# Autodesk Inventor assembly: Catapult Launcher
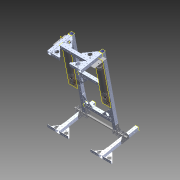
[picture p0: Inventor's stored thumbnail of the model, 180x180]
Saved by Autodesk Inventor 2014 (Build 180170000, 170)
## iProperties
Created: 2014-01-17
Part Number: Catapult Launcher
Document SubType Name: Assembly
Designer: Andrew Toennies
Mass: 1552.27 g
Surface Area: 5150.08 cm^2
Volume: 383.1 cm^3
Density: 4.05187 g/cm^3
Author: Andrew Toennies
## Documents named in this file (14)
- C:\Users\Andrew Toennies\Documents\GitHub\2014buildCAD\New Shooter\Catapult Launcher.iam
- C:\Users\Andrew Toennies\Documents\GitHub\2014buildCAD\New Shooter\Vex Pro 1x1 rectangular tubing 7 in length.ipt
- C:\Users\Andrew Toennies\Documents\GitHub\2014buildCAD\New Shooter\Vex Pro Side Bearing Gusset - OUT OF STOCK 1192014.ipt
- C:\Users\Andrew Toennies\Documents\GitHub\2014buildCAD\New Shooter\Vex Pro Corner Gusset - IN STOCK 1192014.ipt
- C:\Users\Andrew Toennies\Documents\GitHub\2014buildCAD\New Shooter\Bearing ID 0.500 Hex OD 1.125.ipt
- C:\Users\Andrew Toennies\Documents\GitHub\2014buildCAD\New Shooter\Shaft (Steel 0.500 Hex).ipt
- C:\Users\Andrew Toennies\Documents\GitHub\2014buildCAD\New Shooter\Vex Pro 1x1 rectangular tubing 27 in length.ipt
- C:\Users\Andrew Toennies\Documents\GitHub\2014buildCAD\New Shooter\Vex Pro 1x1 rectangular tubing 3 in length.ipt
- C:\Users\Andrew Toennies\Documents\GitHub\2014buildCAD\New Shooter\Vex Pro 1x1 rectangular tubing 11 in length.ipt
- C:\Users\Andrew Toennies\Documents\GitHub\2014buildCAD\New Shooter\1.5 in bore 6 in stroke cylinder - BIMBA\176-DP(D-229)(F,D-231-1).iam
- C:\Users\Andrew Toennies\Documents\GitHub\2014buildCAD\New Shooter\Aluminum Plate (0.125).ipt
- C:\Users\Andrew Toennies\Documents\GitHub\2014buildCAD\New Shooter\1.5 in bore 6 in stroke cylinder - BIMBA\D-14826.ipt
- C:\Users\Andrew Toennies\Documents\GitHub\2014buildCAD\New Shooter\1.5 in bore 6 in stroke cylinder - BIMBA\D-9969.ipt
- C:\Users\Andrew Toennies\Documents\GitHub\2014buildCAD\New Shooter\Vex Pro End Bearing Mount - IN STOCK 1192014.ipt
## Components (44 placed, 13 different names)
1. Shaft (Steel 0.500 Hex):1 — Mate:34, Mate:35, Flush:25, Mate:227, Mate:228
2. Vex Pro 1x1 rectangular tubing 11 in length:3 — Flush:38, Mate:237, Mate:238, Mate:240, Flush:39, Flush:40
3. Vex Pro Corner Gusset - IN STOCK 1192014:9 — Mate:238, Mate:239, Flush:40
4. Vex Pro Corner Gusset - IN STOCK 1192014:10 — Mate:240, Mate:241, Flush:39
5. Vex Pro Corner Gusset - IN STOCK 1192014:11 — Mate:243, Flush:43, Mate:244
6. Vex Pro Corner Gusset - IN STOCK 1192014:12 — Mate:248, Mate:249, Flush:44
7. Vex Pro Corner Gusset - IN STOCK 1192014:13 — Mate:252, Mate:253, Flush:46
8. Vex Pro Corner Gusset - IN STOCK 1192014:14 — Mate:250, Mate:251, Flush:45
9. Vex Pro 1x1 rectangular tubing 7 in length:1 — Flush:1, Flush:2, Mate:8, Mate:11, Mate:20, Mate:21, Mate:22, Mate:23, Mate:24, Mate:25, Mate:195, Flush:32, Flush:33, Flush:34, Flush:35
10. Vex Pro 1x1 rectangular tubing 7 in length:2 — Flush:1, Flush:2, Mate:3, Mate:5, Mate:14, Mate:15, Mate:16, Mate:17, Mate:18, Mate:19, Mate:123, Mate:188, Mate:195, Flush:25, Flush:28, Flush:29, Flush:30, Flush:31
11. Vex Pro Side Bearing Gusset - OUT OF STOCK 1192014:1 — Mate:3, Mate:26, Mate:27, Flush:28, Flush:29
12. Vex Pro Side Bearing Gusset - OUT OF STOCK 1192014:2 — Mate:5, Mate:28, Mate:29, Flush:30, Flush:31
13. Vex Pro Side Bearing Gusset - OUT OF STOCK 1192014:3 — Mate:11, Mate:32, Mate:33, Flush:32, Flush:33
14. Vex Pro Side Bearing Gusset - OUT OF STOCK 1192014:4 — Mate:8, Mate:30, Mate:31, Flush:34, Flush:35
15. Vex Pro Corner Gusset - IN STOCK 1192014:1 — Mate:17, Mate:18, Mate:19, Flush:18
16. Vex Pro Corner Gusset - IN STOCK 1192014:2 — Mate:14, Mate:15, Mate:16
17. Vex Pro Corner Gusset - IN STOCK 1192014:3 — Mate:20, Mate:21, Mate:22
18. Vex Pro Corner Gusset - IN STOCK 1192014:4 — Mate:23, Mate:24, Mate:25
19. Bearing ID 0.500 Hex OD 1.125:1 — Mate:28, Mate:29, Flush:3, Flush:5
20. Bearing ID 0.500 Hex OD 1.125:2 — Mate:26, Mate:27, Flush:3, Mate:34, Mate:35
21. Bearing ID 0.500 Hex OD 1.125:3 — Mate:30, Mate:31, Flush:4
22. Bearing ID 0.500 Hex OD 1.125:4 — Mate:32, Mate:33, Flush:4, Flush:5, Mate:69
23. Vex Pro 1x1 rectangular tubing 11 in length:1 — Mate:191, Flush:42, Mate:250, Mate:253, Flush:46
24. Vex Pro 1x1 rectangular tubing 11 in length:2 — Flush:41, Mate:242, Mate:243, Flush:43, Mate:246, Mate:248, Flush:44
25. D-9969:1 — Mate:164, Mate:165, Mate:166, Mate:198, Flush:36
26. D-14826:1 — Mate:164, Mate:169, Mate:170, Flush:37, Mate:247
27. Vex Pro End Bearing Mount - IN STOCK 1192014:4 — Mate:229, Mate:230, Mate:231, Mate:232, Mate:246
28. Vex Pro End Bearing Mount - IN STOCK 1192014:3 — Mate:217, Mate:218, Mate:219, Mate:220, Mate:221
29. Vex Pro End Bearing Mount - IN STOCK 1192014:2 — Mate:233, Mate:234, Mate:235, Mate:236, Mate:245
30. Vex Pro End Bearing Mount - IN STOCK 1192014:1 — Mate:222, Mate:223, Mate:224, Mate:225, Mate:226
31. Vex Pro 1x1 rectangular tubing 27 in length:3 — Mate:198, Mate:229, Mate:230, Mate:231, Mate:233, Mate:234, Mate:235, Flush:27, Flush:36, Flush:41, Mate:242, Mate:244, Mate:251, Flush:45
32. Vex Pro 1x1 rectangular tubing 27 in length:2 — Mate:188, Mate:191, Mate:212, Mate:213, Mate:219, Mate:220, Mate:221, Mate:224, Mate:225, Mate:226, Flush:26, Flush:37, Flush:42, Mate:247, Mate:249, Mate:252
33. Bearing ID 0.500 Hex OD 1.125:5 — Mate:80, Mate:222, Mate:223, Mate:228
34. Bearing ID 0.500 Hex OD 1.125:6 — Mate:80, Mate:217, Mate:218, Mate:227
35. Bearing ID 0.500 Hex OD 1.125:7 — Mate:68, Mate:69, Mate:236, Mate:245
36. Bearing ID 0.500 Hex OD 1.125:8 — Mate:68, Mate:232
37. 176-DP(D-229)(F,D-231-1):1 [sub-assembly] — Mate:153, Mate:154, Mate:155, Mate:165, Mate:166, Mate:171
38. 176-DP(D-229)(F,D-231-1):2 [sub-assembly] — Mate:156, Mate:167, Mate:168, Mate:169, Mate:170, Mate:171
39. Aluminum Plate (0.125):1 — Mate:153, Mate:154, Mate:155, Mate:159, Flush:24
40. Aluminum Plate (0.125):2 — Mate:156, Mate:160, Mate:167, Mate:168, Flush:24, Mate:213
41. Vex Pro 1x1 rectangular tubing 3 in length:2 — Mate:121, Flush:14, Mate:122, Flush:19, Mate:159, Flush:27, Mate:241
42. Vex Pro 1x1 rectangular tubing 3 in length:1 — Flush:13, Mate:118, Mate:119, Mate:120, Mate:123, Flush:19, Mate:160, Mate:212, Flush:26, Flush:38, Mate:237, Mate:239
43. Vex Pro Corner Gusset - IN STOCK 1192014:8 — Flush:13, Mate:118, Mate:119, Mate:120, Flush:17, Flush:18
44. Vex Pro Corner Gusset - IN STOCK 1192014:6 — Mate:121, Flush:14, Mate:122, Flush:17
## Relationships (125: Mate 92, Flush 33)
- Flush:1: Vex Pro 1x1 rectangular tubing 7 in length:1 ↔ Vex Pro 1x1 rectangular tubing 7 in length:2
- Flush:2: Vex Pro 1x1 rectangular tubing 7 in length:1 ↔ Vex Pro 1x1 rectangular tubing 7 in length:2
- Mate:3: Vex Pro 1x1 rectangular tubing 7 in length:2 ↔ Vex Pro Side Bearing Gusset - OUT OF STOCK 1192014:1
- Mate:5: Vex Pro 1x1 rectangular tubing 7 in length:2 ↔ Vex Pro Side Bearing Gusset - OUT OF STOCK 1192014:2
- Mate:8: Vex Pro 1x1 rectangular tubing 7 in length:1 ↔ Vex Pro Side Bearing Gusset - OUT OF STOCK 1192014:4
- Mate:11: Vex Pro 1x1 rectangular tubing 7 in length:1 ↔ Vex Pro Side Bearing Gusset - OUT OF STOCK 1192014:3
- Mate:14: Vex Pro 1x1 rectangular tubing 7 in length:2 ↔ Vex Pro Corner Gusset - IN STOCK 1192014:2
- Mate:15: Vex Pro 1x1 rectangular tubing 7 in length:2 ↔ Vex Pro Corner Gusset - IN STOCK 1192014:2
- Mate:16: Vex Pro 1x1 rectangular tubing 7 in length:2 ↔ Vex Pro Corner Gusset - IN STOCK 1192014:2
- Mate:17: Vex Pro 1x1 rectangular tubing 7 in length:2 ↔ Vex Pro Corner Gusset - IN STOCK 1192014:1
- Mate:18: Vex Pro 1x1 rectangular tubing 7 in length:2 ↔ Vex Pro Corner Gusset - IN STOCK 1192014:1
- Mate:19: Vex Pro 1x1 rectangular tubing 7 in length:2 ↔ Vex Pro Corner Gusset - IN STOCK 1192014:1
- Mate:20: Vex Pro 1x1 rectangular tubing 7 in length:1 ↔ Vex Pro Corner Gusset - IN STOCK 1192014:3
- Mate:21: Vex Pro 1x1 rectangular tubing 7 in length:1 ↔ Vex Pro Corner Gusset - IN STOCK 1192014:3
- Mate:22: Vex Pro 1x1 rectangular tubing 7 in length:1 ↔ Vex Pro Corner Gusset - IN STOCK 1192014:3
- Mate:23: Vex Pro 1x1 rectangular tubing 7 in length:1 ↔ Vex Pro Corner Gusset - IN STOCK 1192014:4
- Mate:24: Vex Pro 1x1 rectangular tubing 7 in length:1 ↔ Vex Pro Corner Gusset - IN STOCK 1192014:4
- Mate:25: Vex Pro 1x1 rectangular tubing 7 in length:1 ↔ Vex Pro Corner Gusset - IN STOCK 1192014:4
- Mate:26: Vex Pro Side Bearing Gusset - OUT OF STOCK 1192014:1 ↔ Bearing ID 0.500 Hex OD 1.125:2
- Mate:27: Vex Pro Side Bearing Gusset - OUT OF STOCK 1192014:1 ↔ Bearing ID 0.500 Hex OD 1.125:2
- Mate:28: Vex Pro Side Bearing Gusset - OUT OF STOCK 1192014:2 ↔ Bearing ID 0.500 Hex OD 1.125:1
- Mate:29: Vex Pro Side Bearing Gusset - OUT OF STOCK 1192014:2 ↔ Bearing ID 0.500 Hex OD 1.125:1
- Flush:3: Bearing ID 0.500 Hex OD 1.125:1 ↔ Bearing ID 0.500 Hex OD 1.125:2
- Mate:30: Vex Pro Side Bearing Gusset - OUT OF STOCK 1192014:4 ↔ Bearing ID 0.500 Hex OD 1.125:3
- Mate:31: Vex Pro Side Bearing Gusset - OUT OF STOCK 1192014:4 ↔ Bearing ID 0.500 Hex OD 1.125:3
- Mate:32: Vex Pro Side Bearing Gusset - OUT OF STOCK 1192014:3 ↔ Bearing ID 0.500 Hex OD 1.125:4
- Mate:33: Vex Pro Side Bearing Gusset - OUT OF STOCK 1192014:3 ↔ Bearing ID 0.500 Hex OD 1.125:4
- Flush:4: Bearing ID 0.500 Hex OD 1.125:3 ↔ Bearing ID 0.500 Hex OD 1.125:4
- Flush:5: Bearing ID 0.500 Hex OD 1.125:1 ↔ Bearing ID 0.500 Hex OD 1.125:4
- Mate:34: Shaft (Steel 0.500 Hex):1 ↔ Bearing ID 0.500 Hex OD 1.125:2
- Mate:35: Shaft (Steel 0.500 Hex):1 ↔ Bearing ID 0.500 Hex OD 1.125:2
- Mate:68: Bearing ID 0.500 Hex OD 1.125:7 ↔ Bearing ID 0.500 Hex OD 1.125:8
- Mate:69: Bearing ID 0.500 Hex OD 1.125:4 ↔ Bearing ID 0.500 Hex OD 1.125:7
- Mate:80: Bearing ID 0.500 Hex OD 1.125:5 ↔ Bearing ID 0.500 Hex OD 1.125:6
- Flush:13: Vex Pro 1x1 rectangular tubing 3 in length:1 ↔ Vex Pro Corner Gusset - IN STOCK 1192014:8
- Mate:118: Vex Pro 1x1 rectangular tubing 3 in length:1 ↔ Vex Pro Corner Gusset - IN STOCK 1192014:8
- Mate:119: Vex Pro 1x1 rectangular tubing 3 in length:1 ↔ Vex Pro Corner Gusset - IN STOCK 1192014:8
- Mate:120: Vex Pro 1x1 rectangular tubing 3 in length:1 ↔ Vex Pro Corner Gusset - IN STOCK 1192014:8
- Mate:121: Vex Pro 1x1 rectangular tubing 3 in length:2 ↔ Vex Pro Corner Gusset - IN STOCK 1192014:6
- Flush:14: Vex Pro 1x1 rectangular tubing 3 in length:2 ↔ Vex Pro Corner Gusset - IN STOCK 1192014:6
- Mate:122: Vex Pro 1x1 rectangular tubing 3 in length:2 ↔ Vex Pro Corner Gusset - IN STOCK 1192014:6
- Flush:17: Vex Pro Corner Gusset - IN STOCK 1192014:8 ↔ Vex Pro Corner Gusset - IN STOCK 1192014:6
- Flush:18: Vex Pro Corner Gusset - IN STOCK 1192014:1 ↔ Vex Pro Corner Gusset - IN STOCK 1192014:8
- Mate:123 (-685.8 mm): Vex Pro 1x1 rectangular tubing 7 in length:2 ↔ Vex Pro 1x1 rectangular tubing 3 in length:1
- Flush:19: Vex Pro 1x1 rectangular tubing 3 in length:2 ↔ Vex Pro 1x1 rectangular tubing 3 in length:1
- Mate:153: 176-DP(D-229)(F,D-231-1):1 ↔ Aluminum Plate (0.125):1
- Mate:154: 176-DP(D-229)(F,D-231-1):1 ↔ Aluminum Plate (0.125):1
- Mate:155: 176-DP(D-229)(F,D-231-1):1 ↔ Aluminum Plate (0.125):1
- Mate:156: 176-DP(D-229)(F,D-231-1):2 ↔ Aluminum Plate (0.125):2
- Mate:159: Aluminum Plate (0.125):1 ↔ Vex Pro 1x1 rectangular tubing 3 in length:2
- Mate:160: Aluminum Plate (0.125):2 ↔ Vex Pro 1x1 rectangular tubing 3 in length:1
- Mate:164: D-9969:1 ↔ D-14826:1
- Mate:165: D-9969:1 ↔ 176-DP(D-229)(F,D-231-1):1
- Mate:166 (3.2131 mm): D-9969:1 ↔ 176-DP(D-229)(F,D-231-1):1
- Mate:167: 176-DP(D-229)(F,D-231-1):2 ↔ Aluminum Plate (0.125):2
- Mate:168: 176-DP(D-229)(F,D-231-1):2 ↔ Aluminum Plate (0.125):2
- Mate:169: D-14826:1 ↔ 176-DP(D-229)(F,D-231-1):2
- Mate:170 (3.2131 mm): D-14826:1 ↔ 176-DP(D-229)(F,D-231-1):2
- Mate:171: 176-DP(D-229)(F,D-231-1):1 ↔ 176-DP(D-229)(F,D-231-1):2
- Flush:24: Aluminum Plate (0.125):1 ↔ Aluminum Plate (0.125):2
- Mate:188 (25.4 mm): Vex Pro 1x1 rectangular tubing 7 in length:2 ↔ Vex Pro 1x1 rectangular tubing 27 in length:2
- Mate:191: Vex Pro 1x1 rectangular tubing 11 in length:1 ↔ Vex Pro 1x1 rectangular tubing 27 in length:2
- Mate:195 (330.2 mm): Vex Pro 1x1 rectangular tubing 7 in length:1 ↔ Vex Pro 1x1 rectangular tubing 7 in length:2
- Flush:25 (-25.4 mm): Shaft (Steel 0.500 Hex):1 ↔ Vex Pro 1x1 rectangular tubing 7 in length:2
- Mate:198: D-9969:1 ↔ Vex Pro 1x1 rectangular tubing 27 in length:3
- Mate:212: Vex Pro 1x1 rectangular tubing 27 in length:2 ↔ Vex Pro 1x1 rectangular tubing 3 in length:1
- Mate:213: Vex Pro 1x1 rectangular tubing 27 in length:2 ↔ Aluminum Plate (0.125):2
- Mate:217: Vex Pro End Bearing Mount - IN STOCK 1192014:3 ↔ Bearing ID 0.500 Hex OD 1.125:6
- Mate:218: Vex Pro End Bearing Mount - IN STOCK 1192014:3 ↔ Bearing ID 0.500 Hex OD 1.125:6
- Mate:219: Vex Pro End Bearing Mount - IN STOCK 1192014:3 ↔ Vex Pro 1x1 rectangular tubing 27 in length:2
- Mate:220: Vex Pro End Bearing Mount - IN STOCK 1192014:3 ↔ Vex Pro 1x1 rectangular tubing 27 in length:2
- Mate:221: Vex Pro End Bearing Mount - IN STOCK 1192014:3 ↔ Vex Pro 1x1 rectangular tubing 27 in length:2
- Mate:222: Vex Pro End Bearing Mount - IN STOCK 1192014:1 ↔ Bearing ID 0.500 Hex OD 1.125:5
- Mate:223: Vex Pro End Bearing Mount - IN STOCK 1192014:1 ↔ Bearing ID 0.500 Hex OD 1.125:5
- Mate:224: Vex Pro End Bearing Mount - IN STOCK 1192014:1 ↔ Vex Pro 1x1 rectangular tubing 27 in length:2
- Mate:225: Vex Pro End Bearing Mount - IN STOCK 1192014:1 ↔ Vex Pro 1x1 rectangular tubing 27 in length:2
- Mate:226: Vex Pro End Bearing Mount - IN STOCK 1192014:1 ↔ Vex Pro 1x1 rectangular tubing 27 in length:2
- Mate:227: Shaft (Steel 0.500 Hex):1 ↔ Bearing ID 0.500 Hex OD 1.125:6
- Mate:228: Shaft (Steel 0.500 Hex):1 ↔ Bearing ID 0.500 Hex OD 1.125:5
- Mate:229: Vex Pro End Bearing Mount - IN STOCK 1192014:4 ↔ Vex Pro 1x1 rectangular tubing 27 in length:3
- Mate:230: Vex Pro End Bearing Mount - IN STOCK 1192014:4 ↔ Vex Pro 1x1 rectangular tubing 27 in length:3
- Mate:231: Vex Pro End Bearing Mount - IN STOCK 1192014:4 ↔ Vex Pro 1x1 rectangular tubing 27 in length:3
- Mate:232: Vex Pro End Bearing Mount - IN STOCK 1192014:4 ↔ Bearing ID 0.500 Hex OD 1.125:8
- Mate:233: Vex Pro End Bearing Mount - IN STOCK 1192014:2 ↔ Vex Pro 1x1 rectangular tubing 27 in length:3
- Mate:234: Vex Pro End Bearing Mount - IN STOCK 1192014:2 ↔ Vex Pro 1x1 rectangular tubing 27 in length:3
- Mate:235: Vex Pro End Bearing Mount - IN STOCK 1192014:2 ↔ Vex Pro 1x1 rectangular tubing 27 in length:3
- Mate:236: Vex Pro End Bearing Mount - IN STOCK 1192014:2 ↔ Bearing ID 0.500 Hex OD 1.125:7
- Flush:26: Vex Pro 1x1 rectangular tubing 27 in length:2 ↔ Vex Pro 1x1 rectangular tubing 3 in length:1
- Flush:27: Vex Pro 1x1 rectangular tubing 27 in length:3 ↔ Vex Pro 1x1 rectangular tubing 3 in length:2
- Flush:28: Vex Pro 1x1 rectangular tubing 7 in length:2 ↔ Vex Pro Side Bearing Gusset - OUT OF STOCK 1192014:1
- Flush:29 (82.55 mm): Vex Pro 1x1 rectangular tubing 7 in length:2 ↔ Vex Pro Side Bearing Gusset - OUT OF STOCK 1192014:1
- Flush:30: Vex Pro 1x1 rectangular tubing 7 in length:2 ↔ Vex Pro Side Bearing Gusset - OUT OF STOCK 1192014:2
- Flush:31 (-82.55 mm): Vex Pro 1x1 rectangular tubing 7 in length:2 ↔ Vex Pro Side Bearing Gusset - OUT OF STOCK 1192014:2
- Flush:32: Vex Pro 1x1 rectangular tubing 7 in length:1 ↔ Vex Pro Side Bearing Gusset - OUT OF STOCK 1192014:3
- Flush:33 (82.55 mm): Vex Pro 1x1 rectangular tubing 7 in length:1 ↔ Vex Pro Side Bearing Gusset - OUT OF STOCK 1192014:3
- Flush:34: Vex Pro 1x1 rectangular tubing 7 in length:1 ↔ Vex Pro Side Bearing Gusset - OUT OF STOCK 1192014:4
- Flush:35 (-82.55 mm): Vex Pro 1x1 rectangular tubing 7 in length:1 ↔ Vex Pro Side Bearing Gusset - OUT OF STOCK 1192014:4
- Flush:36: D-9969:1 ↔ Vex Pro 1x1 rectangular tubing 27 in length:3
- Flush:37: D-14826:1 ↔ Vex Pro 1x1 rectangular tubing 27 in length:2
- Flush:38: Vex Pro 1x1 rectangular tubing 11 in length:3 ↔ Vex Pro 1x1 rectangular tubing 3 in length:1
- Mate:237: Vex Pro 1x1 rectangular tubing 11 in length:3 ↔ Vex Pro 1x1 rectangular tubing 3 in length:1
- Mate:238: Vex Pro 1x1 rectangular tubing 11 in length:3 ↔ Vex Pro Corner Gusset - IN STOCK 1192014:9
- Mate:239: Vex Pro Corner Gusset - IN STOCK 1192014:9 ↔ Vex Pro 1x1 rectangular tubing 3 in length:1
- Mate:240: Vex Pro 1x1 rectangular tubing 11 in length:3 ↔ Vex Pro Corner Gusset - IN STOCK 1192014:10
- Mate:241: Vex Pro Corner Gusset - IN STOCK 1192014:10 ↔ Vex Pro 1x1 rectangular tubing 3 in length:2
- Flush:39: Vex Pro 1x1 rectangular tubing 11 in length:3 ↔ Vex Pro Corner Gusset - IN STOCK 1192014:10
- Flush:40: Vex Pro 1x1 rectangular tubing 11 in length:3 ↔ Vex Pro Corner Gusset - IN STOCK 1192014:9
- Flush:41: Vex Pro 1x1 rectangular tubing 11 in length:2 ↔ Vex Pro 1x1 rectangular tubing 27 in length:3
- Mate:242: Vex Pro 1x1 rectangular tubing 11 in length:2 ↔ Vex Pro 1x1 rectangular tubing 27 in length:3
- Flush:42: Vex Pro 1x1 rectangular tubing 11 in length:1 ↔ Vex Pro 1x1 rectangular tubing 27 in length:2
- Mate:243: Vex Pro Corner Gusset - IN STOCK 1192014:11 ↔ Vex Pro 1x1 rectangular tubing 11 in length:2
- Flush:43: Vex Pro Corner Gusset - IN STOCK 1192014:11 ↔ Vex Pro 1x1 rectangular tubing 11 in length:2
- Mate:244: Vex Pro Corner Gusset - IN STOCK 1192014:11 ↔ Vex Pro 1x1 rectangular tubing 27 in length:3
- Mate:245: Vex Pro End Bearing Mount - IN STOCK 1192014:2 ↔ Bearing ID 0.500 Hex OD 1.125:7
- Mate:246 (6.35 mm): Vex Pro 1x1 rectangular tubing 11 in length:2 ↔ Vex Pro End Bearing Mount - IN STOCK 1192014:4
- Mate:247: D-14826:1 ↔ Vex Pro 1x1 rectangular tubing 27 in length:2
- Mate:248: Vex Pro Corner Gusset - IN STOCK 1192014:12 ↔ Vex Pro 1x1 rectangular tubing 11 in length:2
- Mate:249: Vex Pro Corner Gusset - IN STOCK 1192014:12 ↔ Vex Pro 1x1 rectangular tubing 27 in length:2
- Flush:44: Vex Pro Corner Gusset - IN STOCK 1192014:12 ↔ Vex Pro 1x1 rectangular tubing 11 in length:2
- Mate:250: Vex Pro Corner Gusset - IN STOCK 1192014:14 ↔ Vex Pro 1x1 rectangular tubing 11 in length:1
- Mate:251: Vex Pro Corner Gusset - IN STOCK 1192014:14 ↔ Vex Pro 1x1 rectangular tubing 27 in length:3
- Flush:45: Vex Pro Corner Gusset - IN STOCK 1192014:14 ↔ Vex Pro 1x1 rectangular tubing 27 in length:3
- Mate:252: Vex Pro Corner Gusset - IN STOCK 1192014:13 ↔ Vex Pro 1x1 rectangular tubing 27 in length:2
- Mate:253: Vex Pro Corner Gusset - IN STOCK 1192014:13 ↔ Vex Pro 1x1 rectangular tubing 11 in length:1
- Flush:46: Vex Pro Corner Gusset - IN STOCK 1192014:13 ↔ Vex Pro 1x1 rectangular tubing 11 in length:1
